# Autodesk Inventor assembly: BB15_block
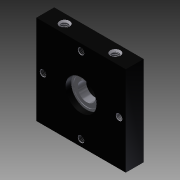
[picture p0: Inventor's stored thumbnail of the model, 180x180]
Saved by Autodesk Inventor 2012 (Build 160160000, 160)
## iProperties
Created: 2012-10-25
Part Number: BB15_block
Document SubType Name: Assembly
Designer: Andrew G. Meyer
Author: Andrew G. Meyer
## Documents named in this file (3)
- C:\Users\Andrew G. Meyer\Documents\Projects\BallBot\macro\CAD\BB15_block.iam
- C:\Users\Andrew G. Meyer\Documents\Projects\BallBot\macro\CAD\BB15_block.ipt
- C:\Users\Andrew G. Meyer\Documents\Projects\BallBot\macro\CAD\P60\BB5-Bearing.ipt
## Components (2 placed, 2 different names)
1. BB15_block:1 — Insert:1
2. BB5-Bearing:1 — Insert:1
## Relationships (1: Insert 1)
- Insert:1: BB15_block:1 ↔ BB5-Bearing:1
